# Autodesk Inventor assembly: !wing
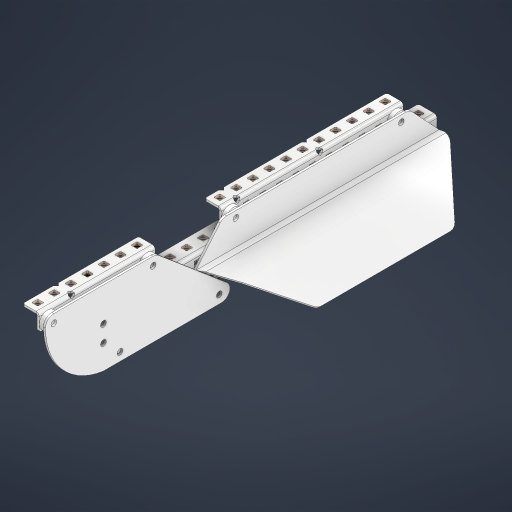
[picture p0: Inventor's stored thumbnail of the model, 512x512]
Saved by Autodesk Inventor 2024 (Build 280153000, 153)
## iProperties
Created: 2023-10-18
Part Number: !wing
Document SubType Name: Assembly
Designer: Averey Ku
Author: Averey Ku
## Documents named in this file (17)
- D:\vex_robotics\hardware\cad\goated_v0.1\chassis\drivebay\wing\!wing.iam
- D:\vex_robotics\hardware\cad\VEX-CAD-Inventor-1.41\Structure\C Channel\Aluminum 1x2x1\Alu C 1x2x1x22.ipt
- D:\vex_robotics\hardware\cad\VEX-CAD-Inventor-1.41\Structure\Angle\Aluminum 1x1\Alu Angle 1x1x7.ipt
- D:\vex_robotics\hardware\cad\VEX-CAD-Inventor-1.41\Structure\Standoff\Standoff .75.ipt
- D:\vex_robotics\hardware\cad\VEX-CAD-Inventor-1.41\Structure\Standoff.ipt
- D:\vex_robotics\hardware\cad\goated_v0.1\chassis\drivebay\custom_parts\sled.ipt
- D:\vex_robotics\hardware\cad\VEX-CAD-Inventor-1.41\Motion\Spacers\Spacer Nylon .375 OD\NSpacer .375 OD x .375.ipt
- D:\vex_robotics\hardware\cad\VEX-CAD-Inventor-1.41\Motion\Spacers\Spacer Nylon .375 OD.ipt
- D:\vex_robotics\hardware\cad\VEX-CAD-Inventor-1.41\Motion\Spacers\Washer Teflon\TWasher .375 OD x .04000.ipt
- D:\vex_robotics\hardware\cad\VEX-CAD-Inventor-1.41\Motion\Spacers\Washer Teflon.ipt
- D:\vex_robotics\hardware\cad\VEX-CAD-Inventor-1.41\Motion\Spacers\Washer Steel\SWasher .375 OD x .015625.ipt
- D:\vex_robotics\hardware\cad\VEX-CAD-Inventor-1.41\Motion\Spacers\Washer Steel.ipt
- D:\vex_robotics\hardware\cad\hardware\.375 OD Aluminum Spacer 0.875.ipt
- D:\vex_robotics\hardware\cad\VEX-CAD-Inventor-1.41\Motion\Spacers\Spacer Nylon .500 OD\NSpacer White .500 OD x .125.ipt
- D:\vex_robotics\hardware\cad\VEX-CAD-Inventor-1.41\Motion\Spacers\Spacer Nylon .500 OD.ipt
- D:\vex_robotics\hardware\cad\VEX-CAD-Inventor-1.41\Structure\Angle\Aluminum 1x1\Alu Angle 1x1x11.ipt
- D:\vex_robotics\hardware\cad\goated_v0.1\chassis\drivebay\wing\custom_parts\wedge.ipt
## Components (24 placed, 11 different names)
1. Alu C 1x2x1x22:1 — Insert:1, Insert:2, Insert:12, Insert:13, Insert:14, Insert:16, Insert:17, Insert:20, Mate:4
2. Alu Angle 1x1x7:1 — Insert:3, Mate:1, Insert:4, Mate:2, Insert:15
3. Standoff .75:1 — Insert:1, Insert:3
4. Standoff .75:2 — Insert:2, Mate:1
5. sled:1 — Insert:4, Mate:2, Insert:5, Mate:3, Insert:18, Insert:19
6. Alu Angle 1x1x7:2 — Insert:5, Mate:3
7. NSpacer .375 OD x .375:1 — Insert:8, Insert:12
8. TWasher .375 OD x .04000:1 — Insert:6, Insert:7
9. TWasher .375 OD x .04000:2 — Insert:7, Insert:8
10. SWasher .375 OD x .015625:1 — Insert:6
11. NSpacer .375 OD x .375:2 — Insert:13
12. TWasher .375 OD x .04000:3
13. TWasher .375 OD x .04000:4
14. SWasher .375 OD x .015625:2
15. .375 OD Aluminum Spacer 0.875:1 — Insert:14
16. NSpacer White .500 OD x .125:1 — Insert:16
17. NSpacer White .500 OD x .125:2 — Insert:18
18. NSpacer White .500 OD x .125:3 — Insert:17
19. NSpacer White .500 OD x .125:4 — Insert:15
20. NSpacer White .500 OD x .125:5 — Insert:19
21. Alu Angle 1x1x11:1 — Insert:20, Mate:4, Insert:21, Mate:5
22. wedge:1 — Insert:21, Mate:5, Insert:22, Insert:23
23. NSpacer White .500 OD x .125:6 — Insert:22
24. NSpacer White .500 OD x .125:7 — Insert:23
## Relationships (28: Insert 23, Mate 5)
- Insert:1: Alu C 1x2x1x22:1 ↔ Standoff .75:1
- Insert:2: Alu C 1x2x1x22:1 ↔ Standoff .75:2
- Insert:3: Alu Angle 1x1x7:1 ↔ Standoff .75:1
- Mate:1: Alu Angle 1x1x7:1 ↔ Standoff .75:2
- Insert:4 (3.175 mm): Alu Angle 1x1x7:1 ↔ sled:1
- Mate:2: Alu Angle 1x1x7:1 ↔ sled:1
- Insert:5 (3.175 mm): sled:1 ↔ Alu Angle 1x1x7:2
- Mate:3: sled:1 ↔ Alu Angle 1x1x7:2
- Insert:6: TWasher .375 OD x .04000:1 ↔ SWasher .375 OD x .015625:1
- Insert:7: TWasher .375 OD x .04000:1 ↔ TWasher .375 OD x .04000:2
- Insert:8: NSpacer .375 OD x .375:1 ↔ TWasher .375 OD x .04000:2
- [Insert]: TWasher .375 OD x .04000:3 ↔ SWasher .375 OD x .015625:2
- [Insert]: TWasher .375 OD x .04000:3 ↔ TWasher .375 OD x .04000:4
- [Insert]: NSpacer .375 OD x .375:2 ↔ TWasher .375 OD x .04000:4
- Insert:12: Alu C 1x2x1x22:1 ↔ NSpacer .375 OD x .375:1
- Insert:13: Alu C 1x2x1x22:1 ↔ NSpacer .375 OD x .375:2
- Insert:14: Alu C 1x2x1x22:1 ↔ .375 OD Aluminum Spacer 0.875:1
- Insert:15: Alu Angle 1x1x7:1 ↔ NSpacer White .500 OD x .125:4
- Insert:16: Alu C 1x2x1x22:1 ↔ NSpacer White .500 OD x .125:1
- Insert:17: Alu C 1x2x1x22:1 ↔ NSpacer White .500 OD x .125:3
- Insert:18: sled:1 ↔ NSpacer White .500 OD x .125:2
- Insert:19: sled:1 ↔ NSpacer White .500 OD x .125:5
- Insert:20 (19.05 mm): Alu C 1x2x1x22:1 ↔ Alu Angle 1x1x11:1
- Mate:4: Alu C 1x2x1x22:1 ↔ Alu Angle 1x1x11:1
- Insert:21 (3.175 mm): Alu Angle 1x1x11:1 ↔ wedge:1
- Mate:5: Alu Angle 1x1x11:1 ↔ wedge:1
- Insert:22: wedge:1 ↔ NSpacer White .500 OD x .125:6
- Insert:23: wedge:1 ↔ NSpacer White .500 OD x .125:7
## Named parameters: d11_d8 = 0 mm, d12_d9 = 0 mm, d13_d10 = 0 mm
